# Autodesk Inventor assembly: stepper_pcb
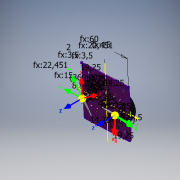
[picture p0: Inventor's stored thumbnail of the model, 180x180]
Saved by Autodesk Inventor 2019 (Build 230136000, 136)
## iProperties
Created: 2018-04-28
Part Number: stepper_pcb
Document SubType Name: Assembly
Designer: Fierl
Author: Fierl
## Documents named in this file (4)
- C:\Users\Fierl\OneDrive - Van Ierland\Documents\Inventor\FlightSim\stepper_pcb.iam
- C:\Users\Fierl\OneDrive - Van Ierland\Documents\Inventor\FlightSim\pcb_board.ipt
- C:\Users\Fierl\OneDrive - Van Ierland\Documents\Inventor\FlightSim\VID26.ipt
- C:\Users\Fierl\OneDrive - Van Ierland\Documents\Inventor\FlightSim\pointer_small.ipt
## Components (5 placed, 3 different names)
1. PCB — Insert:2, Insert:3, Insert:4, Insert:5
2. VID26:3 — Rotational:2, Insert:4, Insert:5
3. VID26:4 — Rotational:1, Insert:2, Insert:3
4. pointer_small:1 — Rotational:1
5. pointer_small:2 — Rotational:2
## Relationships (6: Insert 4, RevoluteJoint 2)
- Rotational:1 [RevoluteJoint]: VID26:4 ↔ pointer_small:1
- Rotational:2 [RevoluteJoint]: VID26:3 ↔ pointer_small:2
- Insert:2: PCB ↔ VID26:4
- Insert:3: PCB ↔ VID26:4
- Insert:4: PCB ↔ VID26:3
- Insert:5: PCB ↔ VID26:3
